# Autodesk Inventor assembly: Rotary_Feedthrough
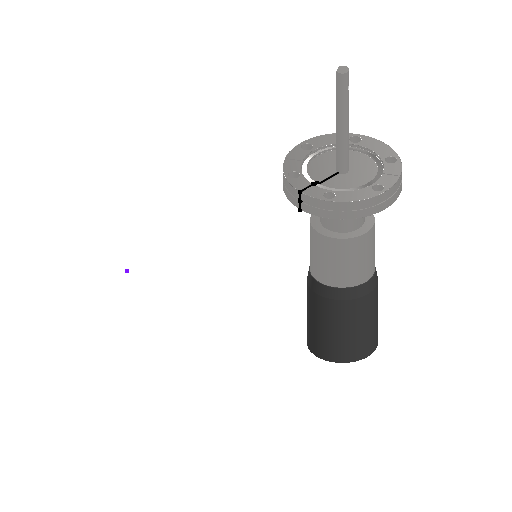
[picture p0: Inventor's stored thumbnail of the model, 512x512]
Saved by Autodesk Inventor 2026.2 (Build 302298000, 298)
## iProperties
Created: 2026-05-26
Part Number: Rotary_Feedthrough
Document SubType Name: Assembly
Designer: zetsu
Author: zetsu
## Documents named in this file (4)
- C:\Users\mzts1\OneDrive - Kyoto University\ドキュメント\蓮尾研究室\3D_CAD\parts\BoronProbe\BoronProbe_5\parts\Rotary_Feedthrough\Rotary_Feedthrough.iam
- C:\Users\mzts1\OneDrive - Kyoto University\ドキュメント\蓮尾研究室\3D_CAD\parts\BoronProbe\BoronProbe_5\parts\Rotary_Feedthrough\ICF-70.ipt
- C:\Users\mzts1\OneDrive - Kyoto University\ドキュメント\蓮尾研究室\3D_CAD\parts\BoronProbe\BoronProbe_5\parts\Rotary_Feedthrough\Rotary_Feedthorough_top.ipt
- C:\Users\mzts1\OneDrive - Kyoto University\ドキュメント\蓮尾研究室\3D_CAD\parts\BoronProbe\BoronProbe_5\parts\Rotary_Feedthrough\Rotary_handle.ipt
## Components (3 placed, 3 different names)
1. ICF-70:1 — メイト:1, メイト:2, 角度:1, メイト:3, メイト:4
2. Rotary_Feedthorough_top:1 — メイト:1, メイト:2, 角度:1
3. Rotary_handle:1 — メイト:3, メイト:4
## Relationships (5: Mate 4, Angle 1)
- メイト:1 [Mate]: ICF-70:1 ↔ Rotary_Feedthorough_top:1
- メイト:2 [Mate]: ICF-70:1 ↔ Rotary_Feedthorough_top:1
- 角度:1 [Angle] (90 deg): ICF-70:1 ↔ Rotary_Feedthorough_top:1
- メイト:3 [Mate]: ICF-70:1 ↔ Rotary_handle:1
- メイト:4 [Mate]: ICF-70:1 ↔ Rotary_handle:1
